# Autodesk Inventor assembly: SM_XA01
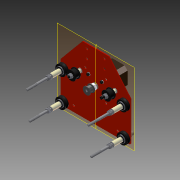
[picture p0: Inventor's stored thumbnail of the model, 180x180]
Saved by Autodesk Inventor 2013 (Build 170138000, 138)
## iProperties
Created: 2012-05-01
Part Number: SM_XA01
Document SubType Name: Assembly
Designer: ERF
Description: X Axis Motor Mount Plate
Stock Number: SM_XA01
Author: ERF
Title: X Axis Motor Mount Plate Assembly
## Documents named in this file (15)
- C:\Users\Brett\Documents\GitHub\BigOko\Assemblies\SM-XA01.iam
- C:\Users\Brett\Documents\GitHub\BigOko\Parts\SM-H04.ipt
- C:\Users\Brett\Documents\GitHub\BigOko\Parts\SM-H01.ipt
- C:\Users\Brett\Documents\GitHub\BigOko\Parts\MSK01-04.ipt
- C:\Users\Brett\Documents\GitHub\BigOko\Parts\SM-H08.ipt
- C:\Users\Brett\Documents\GitHub\BigOko\Parts\SM-S01.ipt
- C:\Users\Brett\Documents\GitHub\BigOko\Parts\MSK01-09.ipt
- C:\Users\Brett\Documents\GitHub\BigOko\Parts\SM-E01.ipt
- C:\Users\Brett\Documents\GitHub\BigOko\Parts\SM-H03.ipt
- C:\Users\Brett\Documents\GitHub\BigOko\Parts\SM-H14.ipt
- C:\Users\Brett\Documents\GitHub\BigOko\Parts\SM-H15.ipt
- C:\Users\Brett\Documents\GitHub\BigOko\Assemblies\MSK01-06A.iam
- C:\Users\Brett\Documents\GitHub\BigOko\Assemblies\MSK01-05A.iam
- C:\Users\Brett\Documents\GitHub\BigOko\bb_parts\Imported Components\shc_90mm\shc_90mm.ipt
- C:\Users\Brett\Documents\GitHub\BigOko\Assemblies\SM-ZA01.iam
## Components (58 placed, 14 different names)
1. SM-ZA01:1 [sub-assembly]
2. SM-H04:1 — Insert:55
3. SM-H01:1 — Insert:26, Insert:28
4. SM-H04:2 — Insert:54
5. SM-H04:3
6. MSK01-04:1 — Insert:5, Insert:8
7. SM-H04:4
8. SM-H01:2 — Insert:25, Insert:27
9. SM-H04:5
10. MSK01-04:2 — Insert:6, Insert:7
11. SM-H04:6
12. SM-H08:1 — Insert:9
13. SM-H08:2 — Insert:10
14. SM-S01:1 — Insert:7, Insert:8, Insert:11, Insert:12, Insert:13, Insert:14, Insert:16, Insert:17, Insert:37, Mate:4, Mate:5, Mate:6, Insert:56, Angle:1, Insert:61, Insert:62, Insert:63, Insert:64
15. MSK01-06A:3 [sub-assembly] — Insert:66, Insert:67
16. MSK01-06A:4 [sub-assembly] — Insert:68, Insert:69
17. MSK01-09:1 — Insert:65
18. MSK01-05A:5 [sub-assembly] — Insert:70, Insert:71
19. MSK01-05A:6 [sub-assembly] — Insert:76, Insert:77
20. MSK01-05A:7 [sub-assembly] — Insert:74, Insert:75
21. MSK01-05A:8 [sub-assembly] — Insert:72, Insert:73
22. SM-E01:1 — Insert:56, Angle:1, Insert:65
23. SM-H03:2 — Insert:5, Insert:78
24. SM-H03:3 — Insert:13, Insert:80
25. SM-H03:4 — Insert:14, Insert:79
26. SM-H03:5 — Insert:6, Insert:81
27. SM-H03:6 — Insert:10, Insert:12
28. SM-H03:7 — Insert:9, Insert:11
29. SM-H03:8 — Insert:76, Insert:85
30. SM-H03:9 — Insert:70, Insert:84
31. SM-H03:10 — Insert:16, Insert:25
32. SM-H03:11 — Insert:17, Insert:26
33. SM-H03:12 — Insert:74, Insert:82
34. SM-H03:13 — Insert:72, Insert:83
35. SM-H03:14 — Insert:27, Insert:68
36. SM-H03:15 — Insert:28, Insert:66
37. SM-H03:16 — Insert:55, Insert:67
38. SM-H03:17 — Insert:54, Insert:69
39. SM-H03:18 — Insert:84
40. SM-H03:19 — Insert:85
41. SM-H03:20 — Insert:83
42. SM-H03:21 — Insert:82
43. SM-H03:22 — Mate:5, Insert:75
44. SM-H03:23 — Mate:6, Insert:73
45. SM-H03:25 — Mate:4, Insert:77
46. SM-H03:26 — Insert:37, Insert:71
47. SM-H15:2 — Insert:57, Insert:64
48. SM-H14:2 — Insert:57
49. SM-H15:3 — Insert:58, Insert:62
50. SM-H14:3 — Insert:58
51. SM-H15:4 — Insert:60, Insert:63
52. SM-H14:4 — Insert:60
53. SM-H15:5 — Insert:59, Insert:61
54. SM-H14:5 — Insert:59
55. shc_90mm:1 — Insert:78
56. shc_90mm:2 — Insert:79
57. shc_90mm:3 — Insert:81
58. shc_90mm:4 — Insert:80
## Relationships (53: Insert 49, Mate 3, Angle 1)
- Insert:5: MSK01-04:1 ↔ SM-H03:2
- Insert:6: MSK01-04:2 ↔ SM-H03:5
- Insert:7: MSK01-04:2 ↔ SM-S01:1
- Insert:8: MSK01-04:1 ↔ SM-S01:1
- Insert:9: SM-H08:1 ↔ SM-H03:7
- Insert:10: SM-H08:2 ↔ SM-H03:6
- Insert:11: SM-S01:1 ↔ SM-H03:7
- Insert:12: SM-S01:1 ↔ SM-H03:6
- Insert:13: SM-S01:1 ↔ SM-H03:3
- Insert:14: SM-S01:1 ↔ SM-H03:4
- Insert:16: SM-S01:1 ↔ SM-H03:10
- Insert:17: SM-S01:1 ↔ SM-H03:11
- Insert:25: SM-H01:2 ↔ SM-H03:10
- Insert:26: SM-H01:1 ↔ SM-H03:11
- Insert:27: SM-H01:2 ↔ SM-H03:14
- Insert:28: SM-H01:1 ↔ SM-H03:15
- Insert:37: SM-S01:1 ↔ SM-H03:26
- Mate:4: SM-S01:1 ↔ SM-H03:25
- Mate:5: SM-S01:1 ↔ SM-H03:22
- Mate:6: SM-S01:1 ↔ SM-H03:23
- Insert:54: SM-H04:2 ↔ SM-H03:17
- Insert:55: SM-H04:1 ↔ SM-H03:16
- Insert:56: SM-S01:1 ↔ SM-E01:1
- Angle:1 (0 deg): SM-S01:1 ↔ SM-E01:1
- Insert:57: SM-H15:2 ↔ SM-H14:2
- Insert:58: SM-H15:3 ↔ SM-H14:3
- Insert:59: SM-H15:5 ↔ SM-H14:5
- Insert:60: SM-H15:4 ↔ SM-H14:4
- Insert:61: SM-S01:1 ↔ SM-H15:5
- Insert:62: SM-S01:1 ↔ SM-H15:3
- Insert:63: SM-S01:1 ↔ SM-H15:4
- Insert:64: SM-S01:1 ↔ SM-H15:2
- Insert:65 (5.08 mm): MSK01-09:1 ↔ SM-E01:1
- Insert:66: MSK01-06A:3 ↔ SM-H03:15
- Insert:67: MSK01-06A:3 ↔ SM-H03:16
- Insert:68: MSK01-06A:4 ↔ SM-H03:14
- Insert:69: MSK01-06A:4 ↔ SM-H03:17
- Insert:70: MSK01-05A:5 ↔ SM-H03:9
- Insert:71: MSK01-05A:5 ↔ SM-H03:26
- Insert:72: MSK01-05A:8 ↔ SM-H03:13
- Insert:73: MSK01-05A:8 ↔ SM-H03:23
- Insert:74: MSK01-05A:7 ↔ SM-H03:12
- Insert:75: MSK01-05A:7 ↔ SM-H03:22
- Insert:76: MSK01-05A:6 ↔ SM-H03:8
- Insert:77: MSK01-05A:6 ↔ SM-H03:25
- Insert:78: SM-H03:2 ↔ shc_90mm:1
- Insert:79: SM-H03:4 ↔ shc_90mm:2
- Insert:80: SM-H03:3 ↔ shc_90mm:4
- Insert:81: SM-H03:5 ↔ shc_90mm:3
- Insert:82: SM-H03:12 ↔ SM-H03:21
- Insert:83: SM-H03:13 ↔ SM-H03:20
- Insert:84: SM-H03:9 ↔ SM-H03:18
- Insert:85: SM-H03:8 ↔ SM-H03:19
